# Autodesk Inventor assembly: WheelAssy
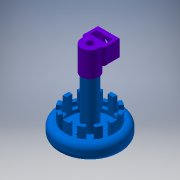
[picture p0: Inventor's stored thumbnail of the model, 180x180]
Saved by Autodesk Inventor 2016 (Build 200138000, 138)
## iProperties
Created: 2015-06-05
Part Number: WheelAssy
Document SubType Name: Assembly
Designer: Erin
Author: Erin
## Documents named in this file (3)
- C:\Users\Erin\Desktop\RDAS v0.2\WheelAssy.iam
- C:\Users\Erin\Desktop\RDAS v0.2\Wheel.ipt
- C:\Users\Erin\Desktop\RDAS v0.2\MotorAttachment.ipt
## Components (2 placed, 2 different names)
1. Wheel:1 — Insert:1
2. MotorAttachment:1 — Insert:1
## Relationships (1: Insert 1)
- Insert:1: Wheel:1 ↔ MotorAttachment:1
